# Autodesk Inventor assembly: wheelbasketleft
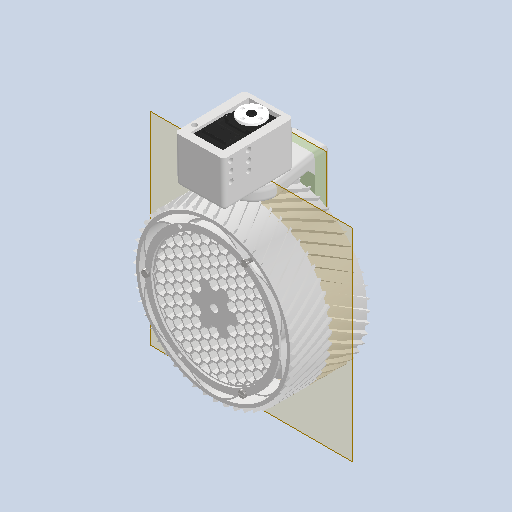
[picture p0: Inventor's stored thumbnail of the model, 512x512]
Saved by Autodesk Inventor 2025.3 (Build 293356000, 356)
## iProperties
Created: 2026-04-12
Part Number: wheelbasketleft
Document SubType Name: Assembly
Designer: ksawe
Author: ksawe
## Documents named in this file (3)
- C:\Users\ksawe\OneDrive\Pulpit\Exomy v1\wersja2\wheelbasketleft.iam
- C:\Users\ksawe\OneDrive\Pulpit\Exomy v1\wersja2\basketleftservo.iam
- C:\Users\ksawe\OneDrive\Pulpit\Exomy v1\wersja2\kolowahacz.iam
## Components (2 placed, 2 different names)
1. basketleftservo:1 [sub-assembly] — Mate:1, Mate:2
2. kolowahacz:1 [sub-assembly] — Mate:1, Mate:2
## Relationships (2: Mate 2)
- Mate:1: basketleftservo:1 ↔ kolowahacz:1
- Mate:2: basketleftservo:1 ↔ kolowahacz:1
